# Autodesk Inventor assembly: varsity wheel
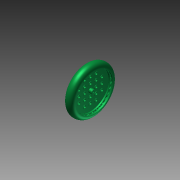
[picture p0: Inventor's stored thumbnail of the model, 180x180]
Saved by Autodesk Inventor 2014 SP1 (Build 180222100, 222)
## iProperties
Created: 2014-02-23
Part Number: varsity wheel
Document SubType Name: Assembly
Designer: Ryan
Author: Ryan
## Documents named in this file (3)
- C:\Users\Ryan\Desktop\sw\toss up 4th robot\drive\varsity wheel.iam
- C:\Users\Ryan\Desktop\sw\lib\Aperture VEX CAD Library\Sprockets\green\High Strength 30-Tooth Sprocket.ipt
- C:\Users\Ryan\Desktop\sw\lib\Super Sonic Sparks VEX CAD Library\Wheels\4'' (Diameter) Wheel With High Traction Tire-Parts\4'' High Traction Tire.ipt
## Components (2 placed, 2 different names)
1. High Strength 30-Tooth Sprocket:1 — Mate:1, Mate:2
2. 4'' High Traction Tire:1 — Mate:1, Mate:2
## Relationships (2: Mate 2)
- Mate:1: High Strength 30-Tooth Sprocket:1 ↔ 4'' High Traction Tire:1
- Mate:2: High Strength 30-Tooth Sprocket:1 ↔ 4'' High Traction Tire:1
